# Autodesk Inventor assembly: elevation_assembly
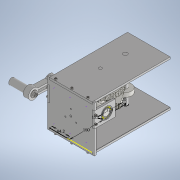
[picture p0: Inventor's stored thumbnail of the model, 180x180]
Saved by Autodesk Inventor 2020 (Build 240168000, 168)
## iProperties
Created: 2020-05-17
Part Number: elevation_assembly
Document SubType Name: Assembly
Designer: Hesekiel
Author: Hesekiel
## Documents named in this file (7)
- C:\Users\Hesekiel\Desktop\Equatorial-Mount-MUM\Mechanika\Mechanizm elewacji Filip\CAD\elevation_assembly.iam
- C:\Users\Hesekiel\Desktop\Equatorial-Mount-MUM\Mechanika\Mechanizm elewacji Filip\CAD\worm_gear.iam
- C:\Users\Hesekiel\Desktop\Equatorial-Mount-MUM\Mechanika\Mechanizm elewacji Filip\CAD\rack_and_pinion.iam
- C:\Users\Hesekiel\Desktop\Equatorial-Mount-MUM\Mechanika\Mechanizm elewacji Filip\CAD\wał_uzębienia.ipt
- C:\Users\Hesekiel\Desktop\Equatorial-Mount-MUM\Mechanika\Mechanizm elewacji Filip\CAD\M6x6_DIN914.ipt
- C:\Users\Hesekiel\Desktop\Equatorial-Mount-MUM\Mechanika\Mechanizm elewacji Filip\CAD\płyta_bazowa_elewacji.iam
- C:\Users\Hesekiel\Desktop\Equatorial-Mount-MUM\Mechanika\Mechanizm elewacji Filip\CAD\wał_półkola.ipt
## Components (7 placed, 6 different names)
1. worm_gear:1 [sub-assembly] — Mate:1, Mate:2, Angle:1, Rotational:5
2. rack_and_pinion:1 [sub-assembly] — Mate:4, Mate:5, Mate:6
3. wał_uzębienia:1 — Mate:1, Mate:2, Mate:4, Rigid:5, Rigid:6
4. M6x6_DIN914:1 — Rigid:6
5. M6x6_DIN914:2 — Rigid:5
6. płyta_bazowa_elewacji:1 [sub-assembly] — Rotational:5, Mate:5, Flush:1
7. wał_półkola:1 — Mate:6, Flush:1
## Relationships (10: Mate 5, WeldJoint 2, Angle 1, RevoluteJoint 1, Flush 1)
- Mate:1: worm_gear:1 ↔ wał_uzębienia:1
- Mate:2: worm_gear:1 ↔ wał_uzębienia:1
- Mate:4: rack_and_pinion:1 ↔ wał_uzębienia:1
- Angle:1 (0 deg): worm_gear:1
- Rigid:5 [WeldJoint]: wał_uzębienia:1 ↔ M6x6_DIN914:2
- Rigid:6 [WeldJoint]: wał_uzębienia:1 ↔ M6x6_DIN914:1
- Rotational:5 [RevoluteJoint]: worm_gear:1 ↔ płyta_bazowa_elewacji:1
- Mate:5: rack_and_pinion:1 ↔ płyta_bazowa_elewacji:1
- Mate:6: rack_and_pinion:1 ↔ wał_półkola:1
- Flush:1: płyta_bazowa_elewacji:1 ↔ wał_półkola:1
